# Autodesk Inventor assembly: CASSING_BAS_MEKANIK
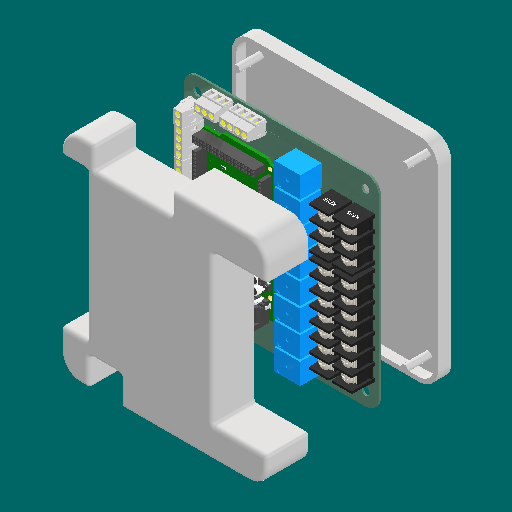
[picture p0: Inventor's stored thumbnail of the model, 512x512]
Saved by Autodesk Inventor 2025.2 (Build 292293000, 293)
## iProperties
Created: 2025-04-28
Part Number: CASSING_BAS_MEKANIK
Document SubType Name: Assembly
Designer: ia088
Author: ia088
## Documents named in this file (4)
- C:\Users\ia088\OneDrive\Dokumen\2matkul_sem4\mikrokontroler\mikro\KRTech\Mekanik\CASSING_BAS_MEKANIK.iam
- C:\Users\ia088\OneDrive\Dokumen\2matkul_sem4\mikrokontroler\mikro\KRTech\Mekanik\BAS_Hardware.iam
- C:\Users\ia088\OneDrive\Dokumen\2matkul_sem4\mikrokontroler\mikro\KRTech\Mekanik\Part_atas.ipt
- C:\Users\ia088\OneDrive\Dokumen\2matkul_sem4\mikrokontroler\mikro\KRTech\Mekanik\Part_bawah.ipt
## Components (3 placed, 3 different names)
1. BAS_Hardware:1 [sub-assembly] — Flush:1, Flush:3, Flush:4, Flush:5, Flush:6
2. Part_atas:1 — Flush:1, Flush:3, Flush:4
3. Part_bawah:1 — Flush:5, Flush:6
## Relationships (5: Flush 5)
- Flush:1: BAS_Hardware:1 ↔ Part_atas:1
- Flush:3: BAS_Hardware:1 ↔ Part_atas:1
- Flush:4: BAS_Hardware:1 ↔ Part_atas:1
- Flush:5: BAS_Hardware:1 ↔ Part_bawah:1
- Flush:6: BAS_Hardware:1 ↔ Part_bawah:1
